# Autodesk Inventor assembly: FO-090.75-NT
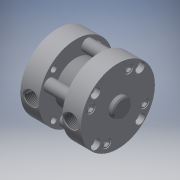
[picture p0: Inventor's stored thumbnail of the model, 180x180]
Saved by Autodesk Inventor 2019.4 (Build 234330000, 330)
## iProperties
Category: PARTsolutions
Company: BIMBA
Created: 2020-02-04
Part Number: FO-090.75-NT
Catalog Web Link: www.cadenas.de
Description: FO, FOD, FOR, FOS-Bimba FLAT-1
Vendor: BIMBA
Document SubType Name: Assembly
Designer: psadmin
Manufacturer: BIMBA
Mass: 52.668 g
Surface Area: 292.615 cm^2
Volume: 52.668 cm^3
Density: 1 g/cm^3
PSOL_IDENT_0: {$CADENAS_DATA\23d-libs\bimba\bimba_brand\bimba_imperial\bimba_full_line\flat_cylinders\fo1\bif_asmt
PSOL_IDENT_1: ab.prj},324 {VTYP=3D},{STYP=ASSTAB},{NB=FO-090.75-NT},{LINA=FO-090.75-NT},{NN=FO, FOD, FOR, FOS},{DA
PSOL_IDENT_2: TE=22.01.2020 09:06:06},{GEOMDATE=12.06.2019 07:36:45},{VERSION=},{LINEID=30},{WBVAR=STROKE,ACTING,M
PSOL_IDENT_3: NTR,MNTF,EE,EEL,TWAB,B,RT,LPHD,G,HR,FO,CRB,FS,M,PP,TO,RM,UM,STPT1,STPT3,STPT4,STPTU1,STPTU3,STPTU4,M
PSOL_IDENT_4: RS,W,CB,TB},{WBNUMERIC=STROKE,EEL}  {NB=FO-090.75-NT},{LINA=FO-090.75-NT},{KT=DUMMY},{PN=FO-090.75-N
PSOL_IDENT_5: T},{PNA=(NO ACCESSORIES)},{PNC=FO-090.75-NT},{BORE=1 1/16\" (09)},{BORE1=1.06250000},{BOREPN=09},{ST
PSOL_IDENT_6: ROKE=0.75},{STROKEMIN=0.12500},{STROKEMAX=16.00000000},{ACTING=},{ACTINGALG='','Double Acting, Singl
PSOL_IDENT_7: e End Rod [FO]', 'D'  , 'Double Acting, Double End Rod [FOD]', 'R', 'Reverse Acting [FOR]', 'S'  ,'S
PSOL_IDENT_8: ingle Acting [FOS]'},{MNTR=},{MNTF=},{MNT=},{MNTALG='','Standard Counterbored Mounting Holes','1','P
PSOL_IDENT_9: ivot Mount','1N','Pivot Mount 90 Deg. from Standard','2','Trunnion Mount, Both Ends','2F','Trunnion
PSOL_IDENT_10: Mount, Front','2R','Trunnion Mount, Rear','3','Threaded Mounting Holes, Both Ends','3F','Threaded Mo
PSOL_IDENT_11: unting Holes, Front','3R','Threaded Mounting Holes, Rear','4','Screw Clearance Holes, Both Ends','4F'
PSOL_IDENT_12: ,'Screw Clearance Holes, Front','4R','Screw Clearance Holes, Rear','5','Nose Mount'},{EEMAX=17.25},{
PSOL_IDENT_13: EE=},{EEALG='','Without Extra Extension','EE','With Extra Extension'},{EEL=0.000},{EELALG=0},{OPLALG=''
PSOL_IDENT_14: ,'Standard Grease Lube','99','Oil Pre-Lube [99]'},{TWAB=},{TWABALG='','Standard Stainless Steel Body'
PSOL_IDENT_15: ,'AB','Thick Walled Aluminum Body [AB]','PB','Composite Body [PB]' },{B=},{BALG='','Without Bumper','
PSOL_IDENT_16: B','Bumper, Both Ends','BR','Bumper, Rear Only','BF','Bumper, Front Only'},{RT=NT},{RTALG='', 'Stand
PSOL_IDENT_17: ard Female Thread 5/16-24 UNF-2B', 'CFT', 'Coarse Female Thread 5/16-18 UNC-2B [CFT]', 'CMT'  , 'Mal
PSOL_IDENT_18: e Rod End (Coarse) 5/16-18 UNC-2B [CMT]', 'MT', 'Male Rod End (Fine) 5/16-24 UNF-2B [MT]', 'NT'  , '
PSOL_IDENT_19: Non-Threaded Rod (Plain Rod) [NT]'},{LPHD=},{LPHDALG='','Standard Pressure Design','D','Low Pressure
PSOL_IDENT_20: Hydraulic Design (250 psi max) [D]'},{G=},{GALG='','Standard Grease Lube','99','Oil Pre-Lube [99]'}
PSOL_IDENT_21: ,{HR=},{HRALG='','N/A'},{HD=},{HDALG='', 'Standard Rear Head', 'HD', 'Heavy Duty Rear Head'},{FO=},{
PSOL_IDENT_22: FOALG='','N/A'},{CRB=},{CRBALG='','Standard Rod Bushing','K','Composite Rod Bushing [K]'},{FS=},{FSA
PSOL_IDENT_23: LG='','Standard Friction Seals','L','Low Friction Seals', 'X', 'Ring Rod Seal'},{FSPNL=},{FSPNX=},{M=
PSOL_IDENT_24: },{MALG='','Without Magnetic Position Sensing','M','With Magnetic Position Sensing [M]','M1','With M
PSOL_IDENT_25: agnetic Position Sensing (Position 1) [M1]','M3','With Magnetic Position Sensing (Position 3) [M3]'
PSOL_IDENT_26: ,'M4','With Magnetic Position Sensing (Position 4) [M4]' },{PB=},{PBALG='','N/A'},{PP=},{PPALG='','S
PSOL_IDENT_27: tandard (ports in line, position #1)','P2','Rotated 90° CW (position #2)','P3','Rotated 180° (positi
PSOL_IDENT_28: on #3)','P4','Rotated 90° CCW (position #4)'},{TO=},{TOALG= '', 'Standard Temp', 'Q'  , 'Low Tempera
PSOL_IDENT_29: ture Operation (-40°F to 200°F)', 'V'  , 'High Temperature Option (0°F to 400°F)' },{S=},{SALG='', '
PSOL_IDENT_30: Without Stainless Steel Fasteners', 'S'  , 'With Stainless Steel Fasteners'},{ST=},{STALG= '' , 'N/A'
PSOL_IDENT_31: },{RM=},{RMALG='', 'Chrome Plated Stainless Steel', 'SR'  , 'Non-Chrome Plated Stainless Steel Rod
PSOL_IDENT_32: [SR]'},{UM=},{STPT1=},{STPT1ALG= '' , 'N/A' },{STPT2=},{STPT2ALG= '' , 'N/A' },{STPT3=},{STPT3ALG= ''
PSOL_IDENT_33: , 'N/A' },{STPT4=},{STPT4ALG= '' , 'N/A' },{UMALG='','Without Magnetic Position Sensing 90°','U','W
PSOL_IDENT_34: ith Magnetic Position Sensing 90° [U]','U1','With Magnetic Position Sensing 90° (Position 1) [U1]','
PSOL_IDENT_35: U3','With Magnetic Position Sensing 90° (Position 3) [U3]'  ,'U4','With Magnetic Position Sensing 90
PSOL_IDENT_36: ° (Position 4) [U4]' },{STPTU1=},{STPTU1ALG= '' , 'N/A' },{STPTU3=},{STPTU3ALG= '' , 'N/A' },{STPTU4=
PSOL_IDENT_37: },{STPTU4ALG= '' , 'N/A' },{U4ALG= ,'U4','With Magnetic Position Sensing 90° (Position 4) [U4]' },{S
PSOL_IDENT_38: OALG='', 'Without Ring Rod Seal', 'X', 'With Ring Rod Seal'},{SO=},{MRS=},{MRSALG='','None ','Z','Me
PSOL_IDENT_39: tallic Rod Scraper [Z]'},{W=},{WALG='', 'Without Wiper', 'W', 'With Wiper'},{Y=},{YALG='', 'Without
PSOL_IDENT_40: Moly-Coat', 'Y', 'With Moly-Coat'},{RP=},{CB=},{TB=},{A=2.00},{B1=0.13},{BA=0.88},{BA1=0.88},{BB=0.0
PSOL_IDENT_41: 0},{BB1=0.94},{BC=0.00},{BD=0.00},{B11=-},{C=1.69},{DD=4},{D=#6},{CPIL=0.15600000},{DC=0.25000000},{
PSOL_IDENT_42: DCP=0.14800000},{DCD=1.68700000},{ES=5/16-24 UNF-2B},{EC=5/16-18 UNC-2B},{ED=0.700},{F=0.50},{G1=0.1
PSOL_IDENT_43: 6},{H=0.44},{HH=},{J=0.50},{K=0.28},{K1=0.28},{K2=0.44},{L=1/8 NPT},{ANGLE=45},{LDP=0.32300000},{LP=
PSOL_IDENT_44: 0.12500000},{LPDP=0.59000000},{TD=1.11200000},{TDDP=0.21800},{TD1=1.10900},{TD2=1.12200},{TDIN=1.062
PSOL_IDENT_45: 00},{LSF=0.00000000},{LSFDP=0.00000000},{BC1=0.88000},{BC2=1.50000},{BC3=2.13000},{BC4=2.75000},{BD1=
PSOL_IDENT_46: 1.38000},{BD2=2.00000},{BD3=2.63000},{BD4=3.25000},{BBB=0.88},{FSADD1=0.37500000},{HDADD1=0.19000000
PSOL_IDENT_47: },{MADD1=0.875},{M1=0.87500000},{M2=0.87500000},{M3=0.87500000},{RL=1.478},{BL=1.066},{LR=0.63},{FSA
PSOL_IDENT_48: DD=0},{HDADD=0},{MADD=0},{ER=},{RL22=0.13},{RL11=0.13000000},{RL1=0.13},{MNTRG=},{MNTRH=},{LG1=0.500
PSOL_IDENT_49: 00000},{LG=0},{RPART=0.316},{AA1=0.13},{AB1=1.50},{AC1=0.75000000},{AD1=1-14 UNS-2A},{AE1=0.998},{AF
PSOL_IDENT_50: 1=0.55},{MM1=0.50},{MM=-},{MM2=0.15},{N=-},{N1=0,25},{NN=0.48},{P1=0.250},{NB1=0.31000000},{P=-},{R=
PSOL_IDENT_51: -},{R1=#6-32 UNC-2B},{R7=#10-32 UNF -28},{Q=-},{Q1=0.19},{S1=-},{S2=0.38},{T=-},{T1=0.25},{U=-},{U1=
PSOL_IDENT_52: 0.25},{W1=-},{W11=0.81},{X=-},{Y1=-},{Z=-},{AA=-},{AB=-},{AC2=0.00},{AC=-},{AD=-},{AE=-},{AF=-},{Z1=
PSOL_IDENT_53: 0.19},{Y11=0.75},{X1=0.25},{DASH=-},{RTPN1=},{RTPN2=NT},{QPN1=},{QPN2=},{EELPN=},{CBALG='','N/A'},{T
PSOL_IDENT_54: BALG='','N/A'},{RPALG='','N/A'},{CBPN=},{TBPN=},{RPPN=},{STPT1PN=},{STPT2PN=},{STPT3PN=},{STPT4PN=},
PSOL_IDENT_55: {RPALG1='','N/A'},{CBALG1='','N/A'},{TBALG1='','N/A'},{CBPN1=},{TBPN1=},{RPPN1=},{CB1=BC-1},{TB1=BT-
PSOL_IDENT_56: 2},{RP1=RP-2},{LR1=0.63},{PPATH=fo1_asmtpl.prj},{MNTRALG='','Standard Counterbored Mounting Holes'
PSOL_IDENT_57: ,'1','Pivot Mount','1N','Pivot Mount 90 Deg. from Standard'   ,'2R','Trunnion Mount, Rear'  ,'3R','T
PSOL_IDENT_58: hreaded Mounting Holes, Rear','4R','Screw Clearance Holes, Rear','6','F Series Interchange, Counterb
PSOL_IDENT_59: ored, Rear [6]' ,'7R','F Series Interchange, Threaded, Rear [7R]'},{MNT2R= ,'2R','Trunnion Mount, Re
PSOL_IDENT_60: ar' },{MNTFALG= '','Standard Counterbored Mounting Holes'    ,'2F','Trunnion Mount, Front'     ,'3F'
PSOL_IDENT_61: ,'Threaded Mounting Holes, Front','4F','Screw Clearance Holes, Front'    ,'5','Nose Mount'      ,'7F'
PSOL_IDENT_62: ,'F Series Interchange, Threaded, Front [7F]'  },{MNT2F= ,'2F','Trunnion Mount, Front' },{MNT5F= ,'5'
PSOL_IDENT_63: ,'Nose Mount'  },{MNTPN=},{MNTPNRH=0},{MNTPNRG=0},{WPN=},{HDPN=},{ASSOPTACC=W},{MATALGHTML=<b>Flat 1
PSOL_IDENT_64: Cylinders:</b><dl><dt>End Caps & Posts:</dt><dd>- Anodized Aluminum</dd><dt> Seals:</dt><dd>- Buna
PSOL_IDENT_65: N </dd><dt>Body:</dt><dd>- 304 Stainless Steel</dd><dt>Bearings:</dt><dd>- Oil Impregnated Bronze</d
PSOL_IDENT_66: d><dt>Rod:</dt><dd>-  303 Stainless Steel</dd></dl>},{STRK2D=0},{X2D=2},{STROKESW=0.750},{EESW=0.000
PSOL_IDENT_67: },{FCD=0},{BCD=0},{RCD=0},{CUSTADD=0.0000},{STPTU1PN=},{STPTU3PN=},{STPTU4PN=},{FOADD=0.000},{NPTF=N
PSOL_IDENT_68: T},{OPLPN=},{GPN=},{TU2CFG=},{TU3CFG=},{TU4CFG=},{MNT4F=,'4F','Screw Clearance Holes, Front'},{NPT=1
PSOL_IDENT_69: /8},{HHFT=0.22},{HHCF=0.22},{HHMT=0.16},{HHMTH=0.16},{HHNPT=0.22},{FTL1=0.700},{NEWPRA=1}
NN: 0.48
NT: Bimba FLAT-1
NB: FO-090.75-NT
NBSYN: $PNC.
LINA: FO-090.75-NT
PN: FO-090.75-NT
PNA: (NO ACCESSORIES)
BORE: 1 1/16" (09)
STROKE: 0.75
ACTING: Double Acting, Single End Rod [FO]
MNTR: Standard Counterbored Mounting Holes
MNTF: Standard Counterbored Mounting Holes
EE: Standard Rod Extension
EEL: 0
TWAB: Standard Stainless Steel Body
B: Without Bumper
RT: Non-Threaded Rod (Plain Rod) [NT]
LPHD: Standard Pressure Design
G: Standard Grease Lube
HR: N/A
FO: N/A
CRB: Standard Rod Bushing
FS: Standard O-Ring Seals
M: Without Magnetic Position Sensing
PP: Standard (ports in line, position #1)
TO: Standard -20° to 200°F (-29° to 95°C)
RM: Chrome Plated Stainless Steel
UM: Without Magnetic Position Sensing 90°
STPT1: N/A
STPT3: N/A
STPT4: N/A
STPTU1: N/A
STPTU3: N/A
STPTU4: N/A
W: Without Wiper
CB: N/A
TB: N/A
A: 2
B1: 0.13
BA: 0.88
BB: 0
BC: 0
BD: 0
B11: -
C: 1.69
DD: 4
D: #6
ES: 5/16-24 UNF-2B
EC: 5/16-18 UNC-2B
ED: 0.7
F: 0.5
G1: 0.16
H: 0.44
J: 0.5
K: 0.28
L: 1/8 NPT
MM: -
MM2: 0.15
N: -
P: -
R: -
Q: -
S1: -
T: -
U: -
W1: -
X: -
Y1: -
Z: -
AA: -
AB: -
AC: -
AD: -
AE: -
AF: -
SUPPLIER: BIMBA
ARTICLENO: FO-090.75-NT
BOMINFO: FO-090.75-NT
CREATOR: CADENAS GmbH
Title: FO-090.75-NT
Author: Cadenas PARTsolutions
Comments: Bimba FLAT-1
## Documents named in this file (9)
- T:\EIT\2020 Infinite Recharge\2020 ROBOT\COMMON PARTS\AIR CYLINDERS\FO-090.75-NT\AIS2018\FO-090_75-NT.iam
- T:\EIT\2020 Infinite Recharge\2020 ROBOT\COMMON PARTS\AIR CYLINDERS\FO-090.75-NT\AIS2018\09-2-0_125-FO1_BM_heads_left-bif.ipt
- T:\EIT\2020 Infinite Recharge\2020 ROBOT\COMMON PARTS\AIR CYLINDERS\FO-090.75-NT\AIS2018\091_061-FO1_BM_tube.ipt
- T:\EIT\2020 Infinite Recharge\2020 ROBOT\COMMON PARTS\AIR CYLINDERS\FO-090.75-NT\AIS2018\09-1NT-0_125-FO1_BM_heads-bif.ipt
- T:\EIT\2020 Infinite Recharge\2020 ROBOT\COMMON PARTS\AIR CYLINDERS\FO-090.75-NT\AIS2018\D-118538-1_422-bif.ipt
- T:\EIT\2020 Infinite Recharge\2020 ROBOT\COMMON PARTS\AIR CYLINDERS\FO-090.75-NT\AIS2018\D-117199-bif.ipt
- T:\EIT\2020 Infinite Recharge\2020 ROBOT\COMMON PARTS\AIR CYLINDERS\FO-090.75-NT\AIS2018\POST1_0625-0_625-bif.ipt
- T:\EIT\2020 Infinite Recharge\2020 ROBOT\COMMON PARTS\AIR CYLINDERS\FO-090.75-NT\AIS2018\FO-090_751_468NT-00_rod-bif.ipt
- T:\EIT\2020 Infinite Recharge\2020 ROBOT\COMMON PARTS\AIR CYLINDERS\FO-090.75-NT\AIS2018\1_06250_311-rod_part0.ipt
## Components (17 placed, 8 different names)
1. 09-2-0_125-FO1_BM_heads_left-bif:1
2. 091_061-FO1_BM_tube:1
3. 09-1NT-0_125-FO1_BM_heads-bif:1 — Insert:2
4. D-118538-1_422-bif:1
5. D-117199-bif:1
6. D-118538-1_422-bif:2
7. D-117199-bif:2
8. D-118538-1_422-bif:3
9. D-117199-bif:3
10. D-118538-1_422-bif:4
11. D-117199-bif:4
12. POST1_0625-0_625-bif:1
13. POST1_0625-0_625-bif:2
14. POST1_0625-0_625-bif:3
15. POST1_0625-0_625-bif:4
16. FO-090_751_468NT-00_rod-bif:1 — Insert:1
17. 1_06250_311-rod_part0:1 — Insert:1, Insert:2
## Relationships (2: Insert 2)
- Insert:1: FO-090_751_468NT-00_rod-bif:1 ↔ 1_06250_311-rod_part0:1
- Insert:2: 09-1NT-0_125-FO1_BM_heads-bif:1 ↔ 1_06250_311-rod_part0:1
